# Autodesk Inventor assembly: ASY Trommel
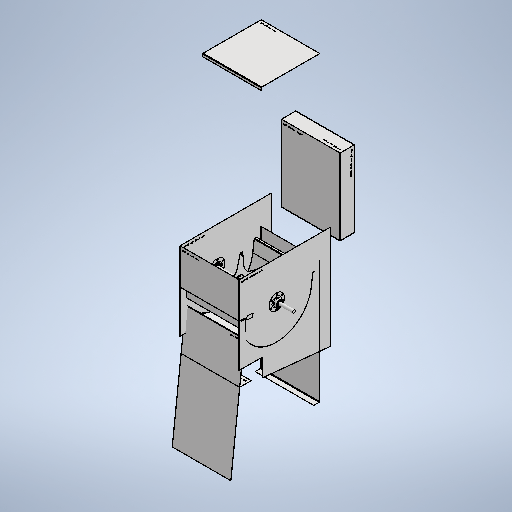
[picture p0: Inventor's stored thumbnail of the model, 512x512]
Saved by Autodesk Inventor 2025 (Build 290162010, 162A)
## iProperties
Created: 2024-08-07
Part Number: ASY Trommel
Document SubType Name: Assembly
Designer: pokla
Author: pokla
## Documents named in this file (21)
- C:\Users\pokla\Documents\Inventor\BSH_Beshkino_bio_tank\ASY Trommel.iam
- C:\Users\pokla\Documents\Inventor\BSH_Beshkino_bio_tank\TRM 011 bottom main.ipt
- C:\Users\pokla\Documents\Inventor\BSH_Beshkino_bio_tank\TRM 012 back main.ipt
- C:\Users\pokla\Documents\Inventor\BSH_Beshkino_bio_tank\TRM 013 top main.ipt
- C:\Users\pokla\Documents\Inventor\BSH_Beshkino_bio_tank\TRM 014 face main.ipt
- C:\Users\pokla\Documents\Inventor\BSH_Beshkino_bio_tank\TRM 015 left board main.ipt
- C:\Users\pokla\Documents\Inventor\BSH_Beshkino_bio_tank\TRM 017 sheet in.ipt
- C:\Users\pokla\Documents\Inventor\BSH_Beshkino_bio_tank\TRM 018 clipper.ipt
- C:\Users\pokla\Documents\Inventor\BSH_Beshkino_bio_tank\TRM 019 tray.ipt
- C:\Users\pokla\Documents\Inventor\BSH_Beshkino_bio_tank\TRM 021 bottom damper.ipt
- C:\Users\pokla\Documents\Inventor\BSH_Beshkino_bio_tank\TRM 022 back damper.ipt
- C:\Users\pokla\Documents\Inventor\BSH_Beshkino_bio_tank\TRM 023 face damper.ipt
- C:\Users\pokla\Documents\Inventor\BSH_Beshkino_bio_tank\TRM 024 top damper.ipt
- C:\Users\pokla\Documents\Inventor\BSH_Beshkino_bio_tank\TRM 025 left board damper.ipt
- C:\Users\pokla\Documents\Inventor\BSH_Beshkino_bio_tank\TRM 026 right board damper.ipt
- C:\Users\pokla\Documents\Inventor\BSH_Beshkino_bio_tank\TRM 027 tromel.ipt
- C:\Users\pokla\Documents\Inventor\BSH_Beshkino_bio_tank\TRM 028 main shaft.ipt
- C:\Users\pokla\Documents\Inventor\BSH_Beshkino_bio_tank\TRM 031 brush.ipt
- C:\Users\pokla\Documents\Inventor\BSH_Beshkino_bio_tank\TRM 016 right board main+.ipt
- C:\Users\pokla\Documents\Inventor\BSH_Beshkino_bio_tank\ASY TRM 020 star.iam
- C:\Users\pokla\Documents\Inventor\BSH_Beshkino_bio_tank\ASY TRM 040 seal.iam
## Components (21 placed, 20 different names)
1. TRM 011 bottom main:1
2. TRM 012 back main:1
3. TRM 013 top main:1
4. TRM 014 face main:1 — Rigid:6, Rigid:17
5. TRM 015 left board main:1 — Mate:2, Angle:1, Mate:5, Flush:1, Mate:7, Mate:8, Rigid:17, Rigid:18
6. TRM 017 sheet in:1 — Rigid:14, Angle:1
7. TRM 018 clipper:1 — Rigid:6
8. TRM 019 tray:1
9. TRM 021 bottom damper:1 — Rigid:8, Rigid:10, Rigid:11, Rigid:12
10. TRM 022 back damper:1 — Rigid:8, Rigid:9
11. TRM 023 face damper:1 — Rigid:10
12. TRM 024 top damper:1 — Rigid:9
13. TRM 025 left board damper:1 — Rigid:11
14. TRM 026 right board damper:1 — Rigid:12
15. TRM 027 tromel:1 — Rigid:14, Mate:4, Mate:5, Mate:9
16. TRM 028 main shaft:1 — Mate:1, Mate:2, Mate:4
17. TRM 031 brush:1 — Flush:1
18. TRM 016 right board main+:1 — Rigid:18, Rigid:20
19. ASY TRM 020 star:1 [sub-assembly]
20. ASY TRM 040 seal:1 [sub-assembly]
21. ASY TRM 040 seal:2 [sub-assembly] — Rigid:20
## Relationships (23: WeldJoint 11, Mate 9, Flush 2, Angle 1)
- Rigid:6 [WeldJoint]: TRM 014 face main:1 ↔ TRM 018 clipper:1
- Rigid:8 [WeldJoint]: TRM 021 bottom damper:1 ↔ TRM 022 back damper:1
- Rigid:9 [WeldJoint]: TRM 022 back damper:1 ↔ TRM 024 top damper:1
- Rigid:10 [WeldJoint]: TRM 021 bottom damper:1 ↔ TRM 023 face damper:1
- Rigid:11 [WeldJoint]: TRM 021 bottom damper:1 ↔ TRM 025 left board damper:1
- Rigid:12 [WeldJoint]: TRM 021 bottom damper:1 ↔ TRM 026 right board damper:1
- Rigid:14 [WeldJoint]: TRM 017 sheet in:1 ↔ TRM 027 tromel:1
- Mate:1: TRM 028 main shaft:1
- Mate:2: TRM 015 left board main:1 ↔ TRM 028 main shaft:1
- [Mate]: TRM 028 main shaft:1 ↔ ASY TRM 020 star:1
- Mate:4: TRM 027 tromel:1 ↔ TRM 028 main shaft:1
- Angle:1 (0 deg): TRM 015 left board main:1 ↔ TRM 017 sheet in:1
- Mate:5: TRM 015 left board main:1 ↔ TRM 027 tromel:1
- Flush:1: TRM 015 left board main:1 ↔ TRM 031 brush:1
- [Mate]: TRM 031 brush:1 ↔ ASY TRM 020 star:1
- [Flush]: TRM 031 brush:1 ↔ ASY TRM 020 star:1
- Mate:7: TRM 015 left board main:1
- Mate:8: TRM 015 left board main:1
- Mate:9: TRM 027 tromel:1
- Rigid:17 [WeldJoint]: TRM 014 face main:1 ↔ TRM 015 left board main:1
- Rigid:18 [WeldJoint] (502 mm): TRM 015 left board main:1 ↔ TRM 016 right board main+:1
- [WeldJoint]: TRM 015 left board main:1 ↔ ASY TRM 040 seal:1
- Rigid:20 [WeldJoint]: TRM 016 right board main+:1 ↔ ASY TRM 040 seal:2
